# Autodesk Inventor assembly: Yassembly
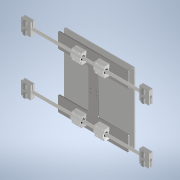
[picture p0: Inventor's stored thumbnail of the model, 180x180]
Saved by Autodesk Inventor 2020.2 (Build 242310000, 310)
## iProperties
Created: 2020-07-30
Part Number: Yassembly
Document SubType Name: Assembly
Designer: JK
Author: JK
## Documents named in this file (4)
- C:\Users\JK\Documents\Inventor\Anet Upgrade\Yassembly.iam
- C:\Users\JK\Documents\Inventor\Anet Upgrade\ycarriage.ipt
- C:\Users\JK\Documents\Inventor\Anet Upgrade\originalbed.ipt
- C:\Users\JK\Documents\Inventor\Anet Upgrade\yrail.iam
## Components (4 placed, 3 different names)
1. ycarriage:1 — Mate:1, Flush:1, Mate:2, Mate:3, Angle:1, Mate:4, Mate:5, Mate:6, Angle:2, Mate:7
2. originalbed:1 — Mate:1, Flush:1
3. yrail:1 [sub-assembly] — Mate:2, Mate:3, Angle:1, Mate:4, Flush:2
4. yrail:2 [sub-assembly] — Mate:5, Mate:6, Angle:2, Flush:2, Mate:7
## Relationships (11: Mate 7, Flush 2, Angle 2)
- Mate:1: ycarriage:1 ↔ originalbed:1
- Flush:1: ycarriage:1 ↔ originalbed:1
- Mate:2: ycarriage:1 ↔ yrail:1
- Mate:3: ycarriage:1 ↔ yrail:1
- Angle:1 (0 deg): ycarriage:1 ↔ yrail:1
- Mate:4: ycarriage:1 ↔ yrail:1
- Mate:5: ycarriage:1 ↔ yrail:2
- Mate:6: ycarriage:1 ↔ yrail:2
- Angle:2 (0 deg): ycarriage:1 ↔ yrail:2
- Flush:2: yrail:1 ↔ yrail:2
- Mate:7: ycarriage:1 ↔ yrail:2
